# Autodesk Inventor assembly: Wing Door
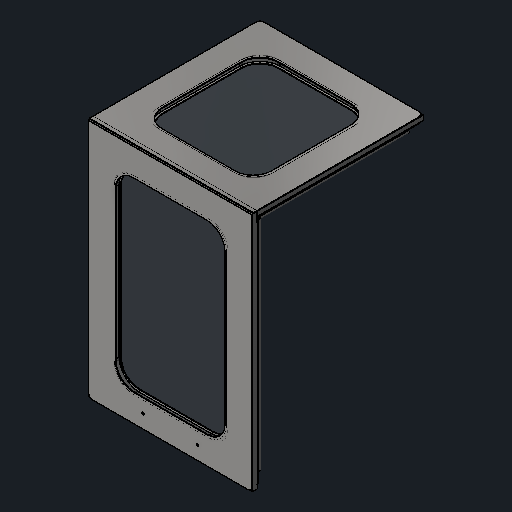
[picture p0: Inventor's stored thumbnail of the model, 512x512]
Saved by Autodesk Inventor 2026.1 (Build 301233020, 233B)
## iProperties
Created: 2025-05-22
Part Number: Wing Door
Document SubType Name: Assembly
Designer: Joshua Eah
Author: Joshua Eah
## Documents named in this file (9)
- C:\Users\JoshuaEah\Documents\GitHub\Voron-0\CAD\Enclosure\Wing Door.iam
- C:\Users\JoshuaEah\Documents\GitHub\Voron-0\CAD\Enclosure\Parts\Foam Tape\Front Door Seal.ipt
- C:\Users\JoshuaEah\Documents\GitHub\Voron-0\CAD\Enclosure\Parts\Metal Panels\Inner Door Panel.ipt
- C:\Users\JoshuaEah\Documents\GitHub\Voron-0\CAD\Enclosure\Parts\Foam Tape\Top Door Seal.ipt
- C:\Users\JoshuaEah\Documents\GitHub\Voron-0\CAD\Enclosure\Parts\Metal Panels\Outer Door Panel.ipt
- C:\Users\JoshuaEah\Documents\GitHub\Voron-0\CAD\Enclosure\Parts\Insulation\Door Panel Front Foam.ipt
- C:\Users\JoshuaEah\Documents\GitHub\Voron-0\CAD\Enclosure\Parts\Insulation\Door Panel Top Foam.ipt
- C:\Users\JoshuaEah\Documents\GitHub\Voron-0\CAD\Enclosure\Parts\Panels\Door Panel Front Panel.ipt
- C:\Users\JoshuaEah\Documents\GitHub\Voron-0\CAD\Enclosure\Parts\Panels\Door Panel Top Panel.ipt
## Components (11 placed, 8 different names)
1. Inner Door Panel:1 — Flush:1, Tangent:1, Tangent:2, Tangent:3, Flush:3, Tangent:7, Tangent:8, Tangent:9, Flush:4, Tangent:10, Tangent:11, Tangent:12, Tangent:13, Flush:5, Tangent:14, Tangent:15, Flush:6, Flush:7, Mate:1, Mate:2, Flush:10, Mate:4, Mate:5, Mate:6, Mate:9, Tangent:16, Tangent:17, Tangent:18
2. Outer Door Panel:1 — Flush:7, Mate:1, Mate:2, Flush:11
3. Front Door Seal:1 — Flush:1, Tangent:1, Tangent:2, Tangent:3
4. Front Door Seal:2 — Flush:4, Tangent:10, Tangent:11, Tangent:12
5. Top Door Seal:1 — Flush:3, Tangent:7, Tangent:8, Tangent:9
6. Top Door Seal:2 — Tangent:13, Flush:5, Tangent:14, Tangent:15
7. Top Door Seal:3 — Flush:6, Tangent:16, Tangent:17, Tangent:18
8. Door Panel Front Foam:1 — Mate:3, Flush:8, Flush:9, Flush:10, Mate:4, Mate:7, Mate:8
9. Door Panel Top Foam:1 — Mate:3, Flush:8, Flush:9, Mate:5, Mate:10, Mate:11
10. Door Panel Front Panel:1 — Mate:6, Mate:7, Mate:8
11. Door Panel Top Panel:1 — Mate:9, Mate:10, Mate:11
## Relationships (36: Tangent 15, Mate 11, Flush 10)
- Flush:1 (20 mm): Inner Door Panel:1 ↔ Front Door Seal:1
- Tangent:1: Inner Door Panel:1 ↔ Front Door Seal:1
- Tangent:2: Inner Door Panel:1 ↔ Front Door Seal:1
- Tangent:3: Inner Door Panel:1 ↔ Front Door Seal:1
- Flush:3 (20 mm): Inner Door Panel:1 ↔ Top Door Seal:1
- Tangent:7: Inner Door Panel:1 ↔ Top Door Seal:1
- Tangent:8: Inner Door Panel:1 ↔ Top Door Seal:1
- Tangent:9: Inner Door Panel:1 ↔ Top Door Seal:1
- Flush:4 (20 mm): Inner Door Panel:1 ↔ Front Door Seal:2
- Tangent:10: Inner Door Panel:1 ↔ Front Door Seal:2
- Tangent:11: Inner Door Panel:1 ↔ Front Door Seal:2
- Tangent:12: Inner Door Panel:1 ↔ Front Door Seal:2
- Tangent:13: Inner Door Panel:1 ↔ Top Door Seal:2
- Flush:5 (20 mm): Inner Door Panel:1 ↔ Top Door Seal:2
- Tangent:14: Inner Door Panel:1 ↔ Top Door Seal:2
- Tangent:15: Inner Door Panel:1 ↔ Top Door Seal:2
- Flush:6 (10 mm): Inner Door Panel:1 ↔ Top Door Seal:3
- Flush:7: Inner Door Panel:1 ↔ Outer Door Panel:1
- Mate:1 (6.35 mm): Inner Door Panel:1 ↔ Outer Door Panel:1
- Mate:2 (6.35 mm): Inner Door Panel:1 ↔ Outer Door Panel:1
- Mate:3: Door Panel Front Foam:1 ↔ Door Panel Top Foam:1
- Flush:8: Door Panel Front Foam:1 ↔ Door Panel Top Foam:1
- Flush:9: Door Panel Front Foam:1 ↔ Door Panel Top Foam:1
- Flush:10: Inner Door Panel:1 ↔ Door Panel Front Foam:1
- Mate:4: Inner Door Panel:1 ↔ Door Panel Front Foam:1
- Mate:5: Inner Door Panel:1 ↔ Door Panel Top Foam:1
- Mate:6: Inner Door Panel:1 ↔ Door Panel Front Panel:1
- Mate:7: Door Panel Front Foam:1 ↔ Door Panel Front Panel:1
- Mate:8: Door Panel Front Foam:1 ↔ Door Panel Front Panel:1
- Mate:9: Inner Door Panel:1 ↔ Door Panel Top Panel:1
- Mate:10: Door Panel Top Foam:1 ↔ Door Panel Top Panel:1
- Mate:11: Door Panel Top Foam:1 ↔ Door Panel Top Panel:1
- Flush:11: Outer Door Panel:1
- Tangent:16: Inner Door Panel:1 ↔ Top Door Seal:3
- Tangent:17: Inner Door Panel:1 ↔ Top Door Seal:3
- Tangent:18: Inner Door Panel:1 ↔ Top Door Seal:3
